# Autodesk Inventor assembly: myrobot
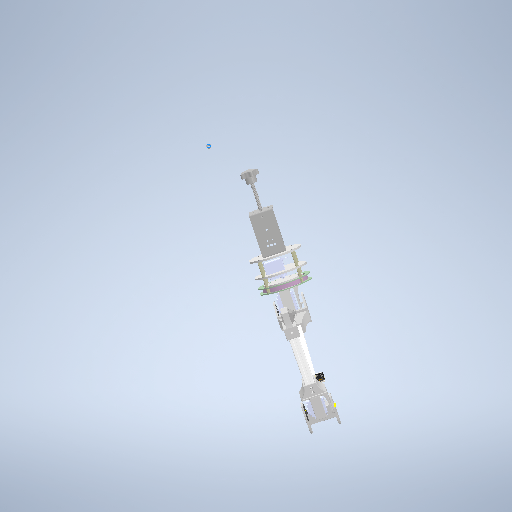
[picture p0: Inventor's stored thumbnail of the model, 512x512]
Saved by Autodesk Inventor 2025 (Build 290162000, 162)
## iProperties
Created: 2024-05-26
Part Number: myrobot
Document SubType Name: Assembly
Designer: hifzh
Author: hifzh
## Documents named in this file (25)
- C:\Users\hifzhil\final_year\Design\TA-Design\part\myrobot.iam
- C:\Users\hifzhil\final_year\Design\TA-Design\part\servo-holder.ipt
- C:\Users\hifzhil\final_year\Design\TA-Design\part\servos.ipt
- C:\Users\hifzhil\final_year\Design\TA-Design\part\horn_connector.ipt
- C:\Users\hifzhil\final_year\Design\TA-Design\part\futaba_horn_35mm_round v1.ipt
- C:\Users\hifzhil\final_year\Design\TA-Design\part\horn-connector2.ipt
- C:\Users\hifzhil\final_year\Design\TA-Design\part\servo-holder2.ipt
- C:\Users\hifzhil\final_year\Design\TA-Design\part\Base_link\bottom-plate.ipt
- C:\Users\hifzhil\final_year\Design\TA-Design\part\Base_link\lower-plate.ipt
- C:\Users\hifzhil\final_year\Design\TA-Design\part\Base_link\6815RS Bearing v1\6815RS Bearing.iam
- C:\Users\hifzhil\final_year\Design\TA-Design\part\Base_link\Ring Plate v1.ipt
- C:\Users\hifzhil\final_year\Design\TA-Design\part\Base_link\M3x10mm Hex Standoff v1.ipt
- C:\Users\hifzhil\final_year\Design\TA-Design\part\Base_link\M3x32mm Hex Standoff v1.ipt
- C:\Users\hifzhil\final_year\Design\TA-Design\part\servo-holder3.ipt
- C:\Users\hifzhil\final_year\Design\TA-Design\part\servo horn 2 v1 v1.ipt
- C:\Users\hifzhil\final_year\Design\TA-Design\part\sg90-servos-v1.ipt
- C:\Users\hifzhil\final_year\Design\TA-Design\part\Board\Seeed Studio XIAO-ESP32-S3-Sense v1\Seeed Studio XIAO-ESP32-S3-Sense.iam
- C:\Users\hifzhil\final_year\Design\TA-Design\part\MR105-2RS.ipt
- C:\Users\hifzhil\final_year\Design\TA-Design\part\almini-18cm.ipt
- C:\Users\hifzhil\final_year\Design\TA-Design\part\almini-26cm.ipt
- C:\Users\hifzhil\final_year\Design\TA-Design\part\Base_link\M3x19mm Hex Standoff v1.ipt
- C:\Users\hifzhil\final_year\Design\TA-Design\part\Base_link\clip_mount.ipt
- C:\Users\hifzhil\final_year\Design\TA-Design\part\table_clip\clip_hole_mur.ipt
- C:\Users\hifzhil\final_year\Design\TA-Design\part\table_clip\holder.ipt
- C:\Users\hifzhil\final_year\Design\TA-Design\part\table_clip\mur_bolt.ipt
## Components (41 placed, 24 different names)
1. servo-holder:1 — Insert:27, Insert:28, Insert:29, Insert:30
2. servos:1 — Insert:27, Rotational:8, Insert:28
3. futaba_horn_35mm_round v1:1 — Rotational:8, Rigid:13
4. horn_connector:1 — Rigid:13, Rigid:14
5. horn-connector2:1 — Rigid:9, Rigid:12
6. futaba_horn_35mm_round v1:2 — Rigid:9, Rotational:7
7. servos:2 — Mate:4, Mate:5, Mate:6, Rotational:7
8. servo-holder2:1 — Mate:4, Mate:5, Mate:6, Rotational:5, Flush:1, Rigid:10
9. lower-plate:1 — Insert:9, Insert:10, Insert:11, Insert:12, Rigid:8
10. 6815RS Bearing:1 [sub-assembly] — Mate:7, Rigid:7, Rigid:8
11. servos:3 — Rigid:5, Insert:23, Insert:36
12. bottom-plate:1 — Rigid:5, Insert:23, Insert:36, Insert:41, Insert:42, Insert:43, Insert:44, Insert:45, Insert:46
13. Ring Plate v1:1 — Mate:7, Insert:3, Insert:4, Insert:5, Insert:6, Rigid:7, Insert:37, Insert:38, Insert:39, Insert:40
14. Ring Plate v1:2 — Insert:7, Insert:8
15. M3x10mm Hex Standoff v1:1 — Insert:3, Insert:8
16. M3x10mm Hex Standoff v1:2 — Insert:4, Insert:7
17. M3x10mm Hex Standoff v1:3 — Insert:6
18. M3x10mm Hex Standoff v1:4 — Insert:5
19. M3x10mm Hex Standoff v1:5 — Insert:9
20. M3x10mm Hex Standoff v1:6 — Insert:10, Insert:30
21. M3x10mm Hex Standoff v1:7 — Insert:11
22. M3x10mm Hex Standoff v1:8 — Insert:12, Insert:29
23. servo-holder3:1 — Insert:24, Insert:25, Insert:26, Rigid:11
24. servo horn 2 v1 v1:1 — Rotational:6
25. sg90-servos-v1:1 — Insert:24, Insert:25, Rotational:6, Insert:26
26. Seeed Studio XIAO-ESP32-S3-Sense:1 [sub-assembly]
27. MR105-2RS:1 — Rotational:5
28. almini-18cm:1 — Rigid:10, Rigid:11
29. almini-26cm:1 — Rigid:12, Rigid:14
30. M3x19mm Hex Standoff v1:1 — Insert:40
31. M3x19mm Hex Standoff v1:2 — Insert:39, Insert:42
32. M3x19mm Hex Standoff v1:3 — Insert:38, Insert:41
33. M3x19mm Hex Standoff v1:4 — Insert:37
34. M3x32mm Hex Standoff v1:1 — Insert:46
35. M3x32mm Hex Standoff v1:2 — Insert:45
36. M3x32mm Hex Standoff v1:3 — Insert:43, Insert:48
37. M3x32mm Hex Standoff v1:4 — Insert:44, Insert:47
38. clip_mount:1 — Insert:47, Insert:48, Insert:49
39. clip_hole_mur:1 — Insert:49, Insert:50
40. holder:1 — Insert:51
41. mur_bolt:1 — Insert:50, Insert:51
## Relationships (52: Insert 34, WeldJoint 9, Mate 4, RevoluteJoint 4, Flush 1)
- Mate:4: servos:2 ↔ servo-holder2:1
- Mate:5: servos:2 ↔ servo-holder2:1
- Mate:6: servos:2 ↔ servo-holder2:1
- Rigid:5 [WeldJoint]: servos:3 ↔ bottom-plate:1
- Mate:7: 6815RS Bearing:1 ↔ Ring Plate v1:1
- Insert:3: Ring Plate v1:1 ↔ M3x10mm Hex Standoff v1:1
- Insert:4: Ring Plate v1:1 ↔ M3x10mm Hex Standoff v1:2
- Insert:5: Ring Plate v1:1 ↔ M3x10mm Hex Standoff v1:4
- Insert:6: Ring Plate v1:1 ↔ M3x10mm Hex Standoff v1:3
- Rigid:7 [WeldJoint] (10 mm): 6815RS Bearing:1 ↔ Ring Plate v1:1
- Insert:7: Ring Plate v1:2 ↔ M3x10mm Hex Standoff v1:2
- Insert:8: Ring Plate v1:2 ↔ M3x10mm Hex Standoff v1:1
- Insert:9: lower-plate:1 ↔ M3x10mm Hex Standoff v1:5
- Insert:10: lower-plate:1 ↔ M3x10mm Hex Standoff v1:6
- Insert:11: lower-plate:1 ↔ M3x10mm Hex Standoff v1:7
- Insert:12: lower-plate:1 ↔ M3x10mm Hex Standoff v1:8
- Rigid:8 [WeldJoint]: lower-plate:1 ↔ 6815RS Bearing:1
- Rigid:9 [WeldJoint]: horn-connector2:1 ↔ futaba_horn_35mm_round v1:2
- Rotational:5 [RevoluteJoint] (-4 mm): servo-holder2:1 ↔ MR105-2RS:1
- Flush:1: servo-holder2:1
- Insert:23: servos:3 ↔ bottom-plate:1
- Insert:24: servo-holder3:1 ↔ sg90-servos-v1:1
- Insert:25: servo-holder3:1 ↔ sg90-servos-v1:1
- Rotational:6 [RevoluteJoint]: servo horn 2 v1 v1:1 ↔ sg90-servos-v1:1
- Insert:26: servo-holder3:1 ↔ sg90-servos-v1:1
- Insert:27: servo-holder:1 ↔ servos:1
- Rigid:10 [WeldJoint]: servo-holder2:1 ↔ almini-18cm:1
- Rotational:7 [RevoluteJoint]: futaba_horn_35mm_round v1:2 ↔ servos:2
- Rigid:11 [WeldJoint]: servo-holder3:1 ↔ almini-18cm:1
- Rigid:12 [WeldJoint] (280 mm): horn-connector2:1 ↔ almini-26cm:1
- Rotational:8 [RevoluteJoint]: servos:1 ↔ futaba_horn_35mm_round v1:1
- Rigid:13 [WeldJoint]: futaba_horn_35mm_round v1:1 ↔ horn_connector:1
- Insert:28: servo-holder:1 ↔ servos:1
- Rigid:14 [WeldJoint]: horn_connector:1 ↔ almini-26cm:1
- Insert:29: servo-holder:1 ↔ M3x10mm Hex Standoff v1:8
- Insert:30: servo-holder:1 ↔ M3x10mm Hex Standoff v1:6
- Insert:36: servos:3 ↔ bottom-plate:1
- Insert:37: Ring Plate v1:1 ↔ M3x19mm Hex Standoff v1:4
- Insert:38: Ring Plate v1:1 ↔ M3x19mm Hex Standoff v1:3
- Insert:39: Ring Plate v1:1 ↔ M3x19mm Hex Standoff v1:2
- Insert:40: Ring Plate v1:1 ↔ M3x19mm Hex Standoff v1:1
- Insert:41: bottom-plate:1 ↔ M3x19mm Hex Standoff v1:3
- Insert:42: bottom-plate:1 ↔ M3x19mm Hex Standoff v1:2
- Insert:43: bottom-plate:1 ↔ M3x32mm Hex Standoff v1:3
- Insert:44: bottom-plate:1 ↔ M3x32mm Hex Standoff v1:4
- Insert:45: bottom-plate:1 ↔ M3x32mm Hex Standoff v1:2
- Insert:46: bottom-plate:1 ↔ M3x32mm Hex Standoff v1:1
- Insert:47: M3x32mm Hex Standoff v1:4 ↔ clip_mount:1
- Insert:48: M3x32mm Hex Standoff v1:3 ↔ clip_mount:1
- Insert:49: clip_mount:1 ↔ clip_hole_mur:1
- Insert:50 (-60 mm): clip_hole_mur:1 ↔ mur_bolt:1
- Insert:51: holder:1 ↔ mur_bolt:1
